# Autodesk Inventor assembly: ridgidity analysis
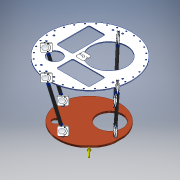
[picture p0: Inventor's stored thumbnail of the model, 180x180]
Saved by Autodesk Inventor 2018 (Build 220112000, 112)
## iProperties
Created: 2019-01-14
Part Number: ridgidity analysis
Document SubType Name: Assembly
Designer: Admin
Author: Admin
## Documents named in this file (12)
- C:\Users\Admin\Documents\Cryostat\CAD\ridgidity analysis.iam
- C:\Users\Admin\Documents\Cryostat\CAD\mini 55K stage.ipt
- C:\Users\Admin\Documents\Cryostat\CAD\2K8 FEET.iam
- C:\Users\Admin\Documents\Cryostat\CAD\2K8 stage mini.ipt
- C:\Users\Admin\Documents\Cryostat\CAD\ridgidity analysis\AIP\FEA\cr7p0y0o0.fins
- C:\Users\Admin\Documents\Cryostat\CAD\ridgidity analysis\AIP\FEA\cr7p0y0o0.fsat
- C:\Users\Admin\Documents\Cryostat\CAD\ridgidity analysis\AIP\FEA\cr7p0y0o0.ftes
- C:\Users\Admin\Documents\Cryostat\CAD\ridgidity analysis\AIP\FEA\cr7p0y0o0.fwiz
- C:\Users\Admin\Documents\Cryostat\CAD\ridgidity analysis\AIP\FEA\cr7q6lls0.fmsh
- C:\Users\Admin\Documents\Cryostat\CAD\ridgidity analysis\AIP\FEA\cr7q6lls1.fres
- C:\Users\Admin\Documents\Cryostat\CAD\ridgidity analysis\AIP\FEA\crgsm8x0g.fmsh
- C:\Users\Admin\Documents\Cryostat\CAD\ridgidity analysis\AIP\FEA\crgsm8x0h.fres
## Components (6 placed, 3 different names)
1. mini 55K stage:1 — Mate:1, Mate:2, Mate:3, Mate:4, Mate:5, Mate:6, Mate:7, Mate:8
2. 2K8 FEET:1 [sub-assembly] — Mate:1, Mate:5, Mate:9, Mate:16
3. 2K8 FEET:2 [sub-assembly] — Mate:3, Mate:8, Mate:12, Mate:13
4. 2K8 FEET:3 [sub-assembly] — Mate:4, Mate:6, Mate:10, Mate:15
5. 2K8 FEET:4 [sub-assembly] — Mate:2, Mate:7, Mate:11, Mate:14
6. 2K8 stage mini:1 — Mate:9, Mate:10, Mate:11, Mate:12, Mate:13, Mate:14, Mate:15, Mate:16
## Relationships (16: Mate 16)
- Mate:1: mini 55K stage:1 ↔ 2K8 FEET:1
- Mate:2: mini 55K stage:1 ↔ 2K8 FEET:4
- Mate:3: mini 55K stage:1 ↔ 2K8 FEET:2
- Mate:4: mini 55K stage:1 ↔ 2K8 FEET:3
- Mate:5: mini 55K stage:1 ↔ 2K8 FEET:1
- Mate:6: mini 55K stage:1 ↔ 2K8 FEET:3
- Mate:7: mini 55K stage:1 ↔ 2K8 FEET:4
- Mate:8: mini 55K stage:1 ↔ 2K8 FEET:2
- Mate:9: 2K8 FEET:1 ↔ 2K8 stage mini:1
- Mate:10: 2K8 FEET:3 ↔ 2K8 stage mini:1
- Mate:11: 2K8 FEET:4 ↔ 2K8 stage mini:1
- Mate:12: 2K8 FEET:2 ↔ 2K8 stage mini:1
- Mate:13: 2K8 FEET:2 ↔ 2K8 stage mini:1
- Mate:14: 2K8 FEET:4 ↔ 2K8 stage mini:1
- Mate:15: 2K8 FEET:3 ↔ 2K8 stage mini:1
- Mate:16: 2K8 FEET:1 ↔ 2K8 stage mini:1
## Named parameters: sa_0 = -314.537, sa_1 = -0, sa_2 = -314.537, sa_3 = -444.822, sa_4 = -0, sa_5 = -3.46961e-11
note: some values were not read from the file. Shown as the stored number, unit unknown: "sa_0", "sa_1", "sa_2", "sa_3", "sa_4", "sa_5".
